# Autodesk Inventor assembly: RollerSmall
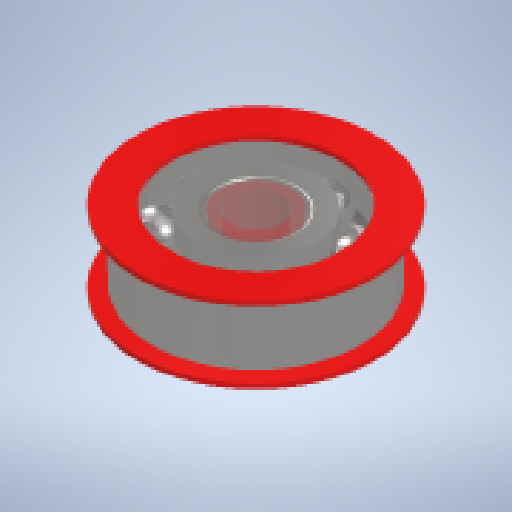
[picture p0: Inventor's stored thumbnail of the model, 512x512]
Saved by Autodesk Inventor 2023 (Build 270158000, 158)
## iProperties
Created: 2023-08-18
Part Number: RollerSmall
Document SubType Name: Assembly
Designer: Felix
Author: Felix
## Documents named in this file (4)
- D:\Programmieren\PineapplePenPlotter\Inventor\try_3\RollerSmall.iam
- C:\Users\Felix\Documents\Inventor\Content Center Files\R2023\en-US\BS 290 SKF(30)\BS 290 SKF - SKF 608.ipt
- D:\Programmieren\PineapplePenPlotter\Inventor\BearingRim.ipt
- D:\Programmieren\PineapplePenPlotter\Inventor\try_3\BearingSpacer.ipt
## Components (4 placed, 3 different names)
1. BS 290 SKF 608:1 — Mate:1, Mate:2, Mate:3, Mate:4, Mate:5, Mate:6
2. BearingRim:1 — Mate:3, Mate:4
3. BearingRim:2 — Mate:1, Mate:2
4. BearingSpacer:1 — Mate:5, Mate:6
## Relationships (6: Mate 6)
- Mate:1: BS 290 SKF 608:1 ↔ BearingRim:2
- Mate:2: BS 290 SKF 608:1 ↔ BearingRim:2
- Mate:3: BS 290 SKF 608:1 ↔ BearingRim:1
- Mate:4: BS 290 SKF 608:1 ↔ BearingRim:1
- Mate:5: BS 290 SKF 608:1 ↔ BearingSpacer:1
- Mate:6: BS 290 SKF 608:1 ↔ BearingSpacer:1
